# Autodesk Inventor assembly: 축
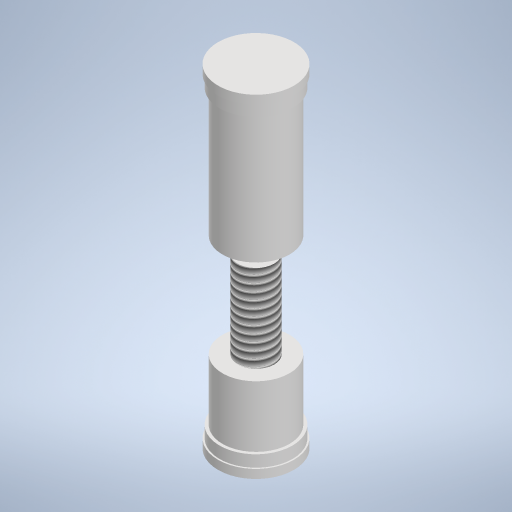
[picture p0: Inventor's stored thumbnail of the model, 512x512]
Saved by Autodesk Inventor 2024 (Build 280153000, 153)
## iProperties
Created: 2023-05-25
Part Number: 축
Document SubType Name: Assembly
Designer: hjcho
Author: hjcho
## Documents named in this file (3)
- C:\Users\hjcho\Desktop\Inventor\축.iam
- C:\Users\hjcho\Desktop\Inventor\축 너트.ipt
- C:\Users\hjcho\Desktop\Inventor\축 볼트.ipt
## Components (2 placed, 2 different names)
1. 축 너트:1 — 메이트:1
2. 축 볼트:1 — 메이트:1
## Relationships (1: Mate 1)
- 메이트:1 [Mate]: 축 너트:1 ↔ 축 볼트:1
